# Autodesk Inventor assembly: modularRICH
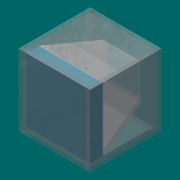
[picture p0: Inventor's stored thumbnail of the model, 180x180]
Saved by Autodesk Inventor 2016 (Build 200138000, 138)
## iProperties
Created: 2015-10-13
Part Number: modularRICH
Document SubType Name: Assembly
Designer: Sawaiz
Author: Sawaiz
## Documents named in this file (5)
- C:\Users\Sawaiz\OneDrive\projects\modularRICH\modularRICH.iam
- C:\Users\Sawaiz\OneDrive\projects\modularRICH\frame\frame.iam
- C:\Users\Sawaiz\OneDrive\projects\modularRICH\mirror\mirror.iam
- C:\Users\Sawaiz\OneDrive\projects\modularRICH\aerogelBlock.ipt
- C:\Users\Sawaiz\OneDrive\projects\modularRICH\fresnelLens.ipt
## Components (4 placed, 4 different names)
1. frame:1 [sub-assembly] — Mate:1, Mate:2, Mate:3, Mate:4, Mate:5, Mate:6
2. mirror:1 [sub-assembly] — Mate:1, Mate:2, Mate:3, Mate:4, Mate:7
3. aerogelBlock:1 — Mate:5, Mate:6, Flush:1, Flush:2, Mate:8
4. fresnelLens:1 — Mate:7, Flush:1, Flush:2, Mate:8
## Relationships (10: Mate 8, Flush 2)
- Mate:1: frame:1 ↔ mirror:1
- Mate:2: frame:1 ↔ mirror:1
- Mate:3: frame:1 ↔ mirror:1
- Mate:4: frame:1 ↔ mirror:1
- Mate:5: frame:1 ↔ aerogelBlock:1
- Mate:6: frame:1 ↔ aerogelBlock:1
- Mate:7: mirror:1 ↔ fresnelLens:1
- Flush:1: aerogelBlock:1 ↔ fresnelLens:1
- Flush:2: aerogelBlock:1 ↔ fresnelLens:1
- Mate:8: aerogelBlock:1 ↔ fresnelLens:1
